# Autodesk Inventor assembly: GE-13048
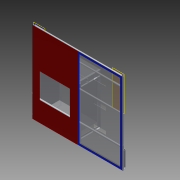
[picture p0: Inventor's stored thumbnail of the model, 180x180]
Saved by Autodesk Inventor 2013 (Build 170138000, 138)
## iProperties
Created: 2013-01-03
Part Number: GE-13048
Document SubType Name: Assembly
Designer: Phillip
Author: Phillip
## Documents named in this file (10)
- E:\Data Folder\FIRST 2013\FIRST KOP\FIRST Arena 2013\Feeder Goal Station\GE-13048.iam
- E:\Data Folder\FIRST 2013\FIRST KOP\FIRST Arena 2013\Feeder Goal Station\GE-13012R.ipt
- E:\Data Folder\FIRST 2013\FIRST KOP\FIRST Arena 2013\Feeder Goal Station\GE-13014.iam
- E:\Data Folder\FIRST 2013\FIRST KOP\FIRST Arena 2013\Feeder Goal Station\GE-13033.iam
- E:\Data Folder\FIRST 2013\FIRST KOP\FIRST Arena 2013\Feeder Goal Station\GE-13032.iam
- E:\Data Folder\FIRST 2013\FIRST KOP\FIRST Arena 2013\Feeder Goal Station\GE-13034.ipt
- E:\Data Folder\FIRST 2013\FIRST KOP\FIRST Arena 2013\Feeder Goal Station\GE-13010.ipt
- E:\Data Folder\FIRST 2013\FIRST KOP\FIRST Arena 2013\Feeder Goal Station\GE-13035.ipt
- E:\Data Folder\FIRST 2013\FIRST KOP\FIRST Arena 2013\Feeder Goal Station\GE-13016.iam
- E:\Data Folder\FIRST 2013\FIRST KOP\FIRST Arena 2013\Feeder Goal Station\FeederTape.ipt
## Components (11 placed, 9 different names)
1. GE-13012R:1 — Flush:1, Mate:9, Flush:2, Flush:5, Flush:10
2. GE-13014:1 [sub-assembly] — Mate:1, Mate:2, Mate:7, Mate:8
3. GE-13033:1 [sub-assembly] — Mate:1, Mate:4, Mate:6, Tangent:1, Tangent:3
4. GE-13033:2 [sub-assembly] — Mate:2, Mate:3, Mate:5, Flush:5, Tangent:2
5. GE-13032:1 [sub-assembly] — Tangent:2, Tangent:3, Mate:12, Flush:10
6. GE-13034:1 — Mate:3, Mate:4, Flush:6
7. GE-13034:2 — Mate:5, Mate:6, Flush:7
8. GE-13010:1 — Flush:8, Flush:9, Mate:11, Flush:11, Flush:12
9. GE-13035:1 — Flush:1, Mate:9, Flush:2, Mate:10, Flush:3, Flush:4, Flush:8, Flush:9, Mate:11
10. GE-13016:1 [sub-assembly] — Mate:7, Mate:8, Mate:10, Flush:3, Flush:4, Mate:12
11. FeederTape:1 — Flush:11, Flush:12
## Relationships (28: Mate 12, Flush 12, Tangent 3, Angle 1)
- Mate:1: GE-13014:1 ↔ GE-13033:1
- Mate:2: GE-13014:1 ↔ GE-13033:2
- Mate:3: GE-13033:2 ↔ GE-13034:1
- Mate:4: GE-13033:1 ↔ GE-13034:1
- Mate:5: GE-13033:2 ↔ GE-13034:2
- Mate:6: GE-13033:1 ↔ GE-13034:2
- Mate:7: GE-13014:1 ↔ GE-13016:1
- Mate:8: GE-13014:1 ↔ GE-13016:1
- Flush:1: GE-13012R:1 ↔ GE-13035:1
- Mate:9: GE-13012R:1 ↔ GE-13035:1
- Flush:2: GE-13012R:1 ↔ GE-13035:1
- Mate:10: GE-13035:1 ↔ GE-13016:1
- Flush:3: GE-13035:1 ↔ GE-13016:1
- Flush:4: GE-13035:1 ↔ GE-13016:1
- Flush:5: GE-13012R:1 ↔ GE-13033:2
- Angle:1 (0 deg)
- Tangent:1: GE-13033:1
- Flush:6 (44.45 mm): GE-13034:1
- Flush:7 (44.45 mm): GE-13034:2
- Flush:8: GE-13010:1 ↔ GE-13035:1
- Flush:9: GE-13010:1 ↔ GE-13035:1
- Mate:11: GE-13010:1 ↔ GE-13035:1
- Tangent:2: GE-13033:2 ↔ GE-13032:1
- Tangent:3: GE-13033:1 ↔ GE-13032:1
- Mate:12: GE-13032:1 ↔ GE-13016:1
- Flush:10 (-19.05 mm): GE-13012R:1 ↔ GE-13032:1
- Flush:11: GE-13010:1 ↔ FeederTape:1
- Flush:12: GE-13010:1 ↔ FeederTape:1
